# Autodesk Inventor assembly: Encoder USD S1-100-B Assy
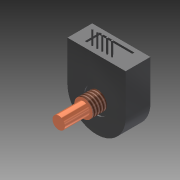
[picture p0: Inventor's stored thumbnail of the model, 180x180]
Saved by Autodesk Inventor 2012 (Build 160160000, 160)
## iProperties
Created: 2012-07-07
Part Number: Encoder USD S1-100-B Assy
Document SubType Name: Assembly
Designer: Programming Team
Author: Programming Team
## Documents named in this file (3)
- C:\Users\Team-2471\Dropbox\Rebound Rumble 2012\Independant Swerves\Imported Components\Encoder USD S1-100-B Assy.iam
- C:\Users\Team-2471\Dropbox\Rebound Rumble 2012\Independant Swerves\Imported Components\USD S1-100-B Housing.ipt
- C:\Users\Team-2471\Dropbox\Rebound Rumble 2012\Independant Swerves\Imported Components\USD S1-100-B Shaft.ipt
## Components (2 placed, 2 different names)
1. USD S1-100-B Housing:1 — Mate:1, Mate:2
2. USD S1-100-B Shaft:1 — Mate:1, Mate:2
## Relationships (2: Mate 2)
- Mate:1: USD S1-100-B Housing:1 ↔ USD S1-100-B Shaft:1
- Mate:2: USD S1-100-B Housing:1 ↔ USD S1-100-B Shaft:1
